# Autodesk Inventor assembly: low_profile_cherry_mx_asm
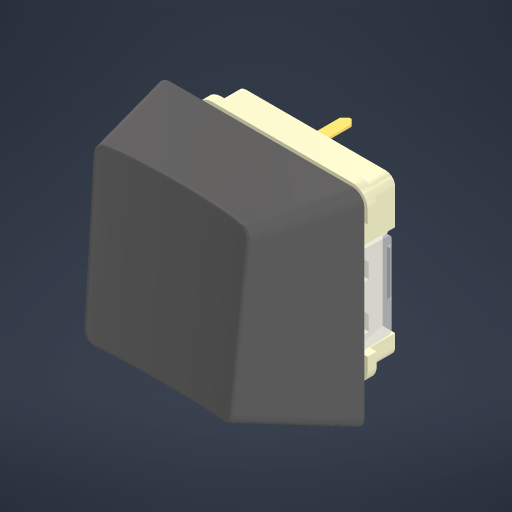
[picture p0: Inventor's stored thumbnail of the model, 512x512]
Saved by Autodesk Inventor 2024 (Build 280153000, 153)
## iProperties
Created: 2026-07-02
Part Number: low_profile_cherry_mx_asm
Document SubType Name: Assembly
Designer: schar
Author: schar
## Documents named in this file (3)
- C:\Users\schar\Projects\Badge\foxbadge\cad\assets\low_profile_cherry_mx_asm.iam
- C:\Users\schar\Projects\Badge\foxbadge\cad\assets\low_profile_cherry_mx.iam
- C:\Users\schar\Projects\Badge\foxbadge\cad\assets\1x1 R2 v8.ipt
## Components (2 placed, 2 different names)
1. low_profile_cherry_mx:1 [sub-assembly] — Mate:1, Mate:2, Mate:3
2. 1x1 R2 v8:1 — Mate:1, Mate:2, Mate:3
## Relationships (3: Mate 3)
- Mate:1: low_profile_cherry_mx:1 ↔ 1x1 R2 v8:1
- Mate:2: low_profile_cherry_mx:1 ↔ 1x1 R2 v8:1
- Mate:3: low_profile_cherry_mx:1 ↔ 1x1 R2 v8:1
